# Autodesk Inventor assembly: PitchAssembly
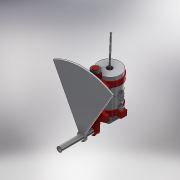
[picture p0: Inventor's stored thumbnail of the model, 180x180]
Saved by Autodesk Inventor 2018 (Build 220112000, 112)
## iProperties
Created: 2018-03-26
Part Number: PitchAssembly
Document SubType Name: Assembly
Designer: mansu
Author: mansu
## Documents named in this file (11)
- F:\OneDrive\Documents\2018 UBC\ELEC 391\Controller\cad\release\PitchAssembly.iam
- F:\OneDrive\Documents\2018 UBC\ELEC 391\Controller\cad\release\Rod3_8in.ipt
- F:\OneDrive\Documents\2018 UBC\ELEC 391\Controller\cad\release\PitchMotor\pitch_motor_flashlight_attached_model.iam
- F:\OneDrive\Documents\2018 UBC\ELEC 391\Controller\cad\release\ShaftArm.ipt
- F:\OneDrive\Documents\2018 UBC\ELEC 391\Controller\cad\release\R1038_ZZ_W Bearing.ipt
- F:\OneDrive\Documents\2018 UBC\ELEC 391\Controller\cad\release\OmegaRing.ipt
- F:\OneDrive\Documents\2018 UBC\ELEC 391\Controller\cad\release\OmegaRingTypeC.ipt
- C:\Users\mansu\Documents\Inventor\Content Center Files\R2018\en-US\AS 1420\AS 1420 - 1973 - M3 x 20.ipt
- C:\Users\mansu\Documents\Inventor\Content Center Files\R2018\en-US\AS 1420\AS 1420 - 1973 - M3 x 14.ipt
- C:\Users\mansu\Documents\Inventor\Content Center Files\R2018\en-US\AS 1474(1)\AS 1474 - M3(1).ipt
- F:\OneDrive\Documents\2018 UBC\ELEC 391\Controller\cad\release\RailBase.ipt
## Components (15 placed, 10 different names)
1. Rod3_8in:1 — Mate:9, Mate:10, Flush:2, Mate:29
2. pitch_motor_flashlight_attached_model:1 [sub-assembly] — Mate:14, Mate:18, Angle:1, Mate:19, Mate:20, Insert:1, Insert:2, Insert:3, Mate:22, Mate:24, Mate:26, Mate:28
3. ShaftArm:1 — Mate:10, Mate:11, Flush:1, Mate:15, Mate:16, Mate:17, Flush:2
4. R1038_ZZ_W Bearing:1 — Mate:11, Flush:1
5. OmegaRing:1 — Mate:14, Mate:15, Mate:17
6. OmegaRingTypeC:1 — Mate:16, Mate:18, Angle:1
7. AS 1420 - Metric M3 x 20:1 — Mate:19, Mate:20, Mate:27
8. AS 1420 - Metric M3 x 20:2 — Insert:1, Mate:21
9. AS 1420 - Metric M3 x 14:1 — Insert:2, Mate:23
10. AS 1420 - Metric M3 x 14:2 — Insert:3, Mate:25
11. AS 1474 - Metric M3:1 — Mate:21, Mate:22
12. AS 1474 - Metric M3:2 — Mate:23, Mate:24
13. AS 1474 - Metric M3:3 — Mate:25, Mate:26
14. AS 1474 - Metric M3:4 — Mate:27, Mate:28
15. RailBase:1 — Mate:29
## Relationships (25: Mate 19, Insert 3, Flush 2, Angle 1)
- Mate:9: Rod3_8in:1
- Mate:10: Rod3_8in:1 ↔ ShaftArm:1
- Mate:11: ShaftArm:1 ↔ R1038_ZZ_W Bearing:1
- Flush:1 (1 mm): ShaftArm:1 ↔ R1038_ZZ_W Bearing:1
- Mate:14: pitch_motor_flashlight_attached_model:1 ↔ OmegaRing:1
- Mate:15: ShaftArm:1 ↔ OmegaRing:1
- Mate:16: ShaftArm:1 ↔ OmegaRingTypeC:1
- Mate:17 (0.1 mm): ShaftArm:1 ↔ OmegaRing:1
- Flush:2: Rod3_8in:1 ↔ ShaftArm:1
- Mate:18: pitch_motor_flashlight_attached_model:1 ↔ OmegaRingTypeC:1
- Angle:1 (0 deg): pitch_motor_flashlight_attached_model:1 ↔ OmegaRingTypeC:1
- Mate:19: pitch_motor_flashlight_attached_model:1 ↔ AS 1420 - Metric M3 x 20:1
- Mate:20: pitch_motor_flashlight_attached_model:1 ↔ AS 1420 - Metric M3 x 20:1
- Insert:1: pitch_motor_flashlight_attached_model:1 ↔ AS 1420 - Metric M3 x 20:2
- Insert:2: pitch_motor_flashlight_attached_model:1 ↔ AS 1420 - Metric M3 x 14:1
- Insert:3: pitch_motor_flashlight_attached_model:1 ↔ AS 1420 - Metric M3 x 14:2
- Mate:21: AS 1420 - Metric M3 x 20:2 ↔ AS 1474 - Metric M3:1
- Mate:22: pitch_motor_flashlight_attached_model:1 ↔ AS 1474 - Metric M3:1
- Mate:23: AS 1420 - Metric M3 x 14:1 ↔ AS 1474 - Metric M3:2
- Mate:24: pitch_motor_flashlight_attached_model:1 ↔ AS 1474 - Metric M3:2
- Mate:25: AS 1420 - Metric M3 x 14:2 ↔ AS 1474 - Metric M3:3
- Mate:26: pitch_motor_flashlight_attached_model:1 ↔ AS 1474 - Metric M3:3
- Mate:27: AS 1420 - Metric M3 x 20:1 ↔ AS 1474 - Metric M3:4
- Mate:28: pitch_motor_flashlight_attached_model:1 ↔ AS 1474 - Metric M3:4
- Mate:29: Rod3_8in:1 ↔ RailBase:1
